# Autodesk Inventor assembly: Z-axis Left Plate
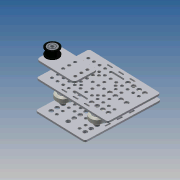
[picture p0: Inventor's stored thumbnail of the model, 180x180]
Saved by Autodesk Inventor 2016 (Build 200138000, 138)
## iProperties
Created: 2015-10-03
Part Number: Z-axis Left Plate
Document SubType Name: Assembly
Designer: Solomon
Author: Solomon
## Documents named in this file (7)
- C:\Users\Solomon\Documents\Inventor\jonathan-printer\Z-axis Left Plate.iam
- C:\Users\Solomon\Documents\Inventor\jonathan-printer\V Slot Part Files\V Slot Plates\Large Build Plate.ipt
- C:\Users\Solomon\Documents\Inventor\jonathan-printer\V Slot Part Files\assembledwheel.iam
- C:\Users\Solomon\Documents\Inventor\jonathan-printer\V Slot Part Files\V Slot Plates\Metric 8mm ACME Block.ipt
- C:\Users\Solomon\Documents\Inventor\jonathan-printer\V Slot Part Files\Pulleys Wheels Bearings\V-Slot Idler Pulley.ipt
- C:\Users\Solomon\Documents\Inventor\jonathan-printer\Imported Components\5mm Bearing SKF 625 (RS 286-7811)\5mm Bearing SKF 625 (RS 286-7811).ipt
- C:\Users\Solomon\Documents\Inventor\jonathan-printer\V Slot Part Files\V Slot Plates\VSlot Idler Pulley Plate.ipt
## Components (12 placed, 6 different names)
1. assembledwheel:1 [sub-assembly] — Angle:8, Mate:7, Mate:8, Angle:15
2. assembledwheel:2 [sub-assembly] — Angle:8, Mate:9, Angle:14
3. assembledwheel:3 [sub-assembly] — Angle:9, Mate:10, Mate:11, Angle:13
4. assembledwheel:4 [sub-assembly] — Mate:6, Mate:12, Mate:13, Angle:12
5. Large Build Plate:2 — Mate:6, Angle:9, Angle:10, Angle:11, Mate:8, Mate:9, Mate:10, Mate:12, Angle:21, Mate:17
6. Large Build Plate:3 — Angle:10, Angle:11, Mate:7, Mate:11, Mate:13, Angle:12, Angle:13, Angle:14, Angle:15, Angle:16, Angle:17, Angle:18, Angle:19, Mate:14, Mate:15, Angle:20, Angle:22
7. Metric 8mm ACME Block:1 — Angle:17, Flush:1, Flush:2, Mate:15
8. Metric 8mm ACME Block:2 — Angle:16, Flush:1, Flush:2, Angle:18, Angle:19, Mate:14
9. V-Slot Idler Pulley:1 — Insert:1, Insert:2
10. 5mm Bearing SKF 625 (RS 286-7811):1 — Insert:1
11. 5mm Bearing SKF 625 (RS 286-7811):2 — Insert:2, Mate:16
12. VSlot Idler Pulley Plate:1 — Mate:16, Angle:20, Angle:21, Angle:22, Mate:17
## Relationships (31: Angle 15, Mate 12, Flush 2, Insert 2)
- Mate:6: assembledwheel:4 ↔ Large Build Plate:2
- Angle:8 (0 deg): assembledwheel:1 ↔ assembledwheel:2
- Angle:9 (0 deg): assembledwheel:3 ↔ Large Build Plate:2
- Angle:10 (0 deg): Large Build Plate:2 ↔ Large Build Plate:3
- Angle:11 (0 deg): Large Build Plate:2 ↔ Large Build Plate:3
- Mate:7: assembledwheel:1 ↔ Large Build Plate:3
- Mate:8: assembledwheel:1 ↔ Large Build Plate:2
- Mate:9: assembledwheel:2 ↔ Large Build Plate:2
- Mate:10: assembledwheel:3 ↔ Large Build Plate:2
- Mate:11: assembledwheel:3 ↔ Large Build Plate:3
- Mate:12: assembledwheel:4 ↔ Large Build Plate:2
- Mate:13: assembledwheel:4 ↔ Large Build Plate:3
- Angle:12 (0 deg): assembledwheel:4 ↔ Large Build Plate:3
- Angle:13 (0 deg): assembledwheel:3 ↔ Large Build Plate:3
- Angle:14 (0 deg): assembledwheel:2 ↔ Large Build Plate:3
- Angle:15 (0 deg): assembledwheel:1 ↔ Large Build Plate:3
- Angle:16 (180 deg): Large Build Plate:3 ↔ Metric 8mm ACME Block:2
- Angle:17 (180 deg): Large Build Plate:3 ↔ Metric 8mm ACME Block:1
- Flush:1: Metric 8mm ACME Block:1 ↔ Metric 8mm ACME Block:2
- Flush:2: Metric 8mm ACME Block:1 ↔ Metric 8mm ACME Block:2
- Angle:18 (0 deg): Large Build Plate:3 ↔ Metric 8mm ACME Block:2
- Angle:19 (0 deg): Large Build Plate:3 ↔ Metric 8mm ACME Block:2
- Mate:14: Large Build Plate:3 ↔ Metric 8mm ACME Block:2
- Mate:15: Large Build Plate:3 ↔ Metric 8mm ACME Block:1
- Insert:1: V-Slot Idler Pulley:1 ↔ 5mm Bearing SKF 625 (RS 286-7811):1
- Insert:2: V-Slot Idler Pulley:1 ↔ 5mm Bearing SKF 625 (RS 286-7811):2
- Mate:16: 5mm Bearing SKF 625 (RS 286-7811):2 ↔ VSlot Idler Pulley Plate:1
- Angle:20 (0 deg): Large Build Plate:3 ↔ VSlot Idler Pulley Plate:1
- Angle:21 (0 deg): Large Build Plate:2 ↔ VSlot Idler Pulley Plate:1
- Angle:22 (0 deg): Large Build Plate:3 ↔ VSlot Idler Pulley Plate:1
- Mate:17: Large Build Plate:2 ↔ VSlot Idler Pulley Plate:1
